# Autodesk Inventor assembly: Elevator
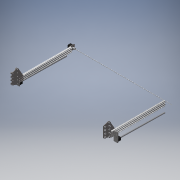
[picture p0: Inventor's stored thumbnail of the model, 180x180]
Saved by Autodesk Inventor 2017 (Build 210142000, 142)
## iProperties
Created: 2016-12-12
Part Number: Elevator
Document SubType Name: Assembly
Designer: umr
Author: umr
## Documents named in this file (21)
- D:\SeniorProject\Models2\Gantry\GantryDown.iam
- D:\SeniorProject\Models2\Gantry\Gantry Plate.ipt
- D:\SeniorProject\Models2\Gantry\M5 Screw with Tee Nut.iam
- D:\SeniorProject\Models2\Gantry\Solid Wheel with Eccentric Spacer Assembly.iam
- D:\SeniorProject\Models2\Gantry\L_Fixer.ipt
- D:\SeniorProject\Models2\Gantry\ScrewDriver.ipt
- D:\SeniorProject\Models2\Gantry\MotorFixer.ipt
- D:\SeniorProject\Models2\Gantry\Elevator Track.ipt
- D:\SeniorProject\Models2\Gantry\Motor.ipt
- D:\SeniorProject\Models2\Gantry\Motor Mount Plate.ipt
- D:\SeniorProject\Models2\Gantry\Driveshaft.ipt
- D:\SeniorProject\Models2\Gantry\5mm x 5mm Flexible Coupling.ipt
- D:\SeniorProject\Models2\Gantry\GT2 20 Tooth Pulley.ipt
- D:\SeniorProject\Models2\Gantry\Gantry Plate_MIR.ipt
- D:\SeniorProject\Models2\Gantry\M5 Screw with Tee Nut_MIR.iam
- D:\SeniorProject\Models2\Gantry\Solid Wheel with Eccentric Spacer Assembly_MIR.iam
- D:\SeniorProject\Models2\Gantry\L_Fixer_MIR.ipt
- D:\SeniorProject\Models2\Gantry\ScrewDriver_MIR.ipt
- D:\SeniorProject\Models2\Gantry\MotorFixer_MIR.ipt
- D:\SeniorProject\Models2\Gantry\Elevator Track_MIR.ipt
- D:\SeniorProject\Models2\Gantry\Motor_MIR.ipt
## Components (62 placed, 20 different names)
1. Gantry Plate:1 — Mate:1, Mate:2, Mate:3, Mate:4, Mate:5, Mate:6, Mate:7, Mate:8, Mate:9, Mate:11, Mate:12, Mate:13, Mate:14, Mate:16, Mate:17, Mate:18, Mate:21, Mate:22, Mate:26, Mate:27, Mate:28, Mate:29, Mate:30, Mate:31, Mate:32, Mate:33, Mate:34, Mate:35, Mate:36, Mate:37, Mate:38, Mate:39, Mate:40, Mate:41, Mate:42, Mate:43
2. M5 Screw with Tee Nut:1 [sub-assembly] — Mate:1, Mate:2
3. M5 Screw with Tee Nut:2 [sub-assembly] — Mate:3, Mate:14
4. M5 Screw with Tee Nut:3 [sub-assembly] — Mate:4, Mate:11
5. M5 Screw with Tee Nut:4 [sub-assembly] — Mate:5, Mate:18
6. M5 Screw with Tee Nut:5 [sub-assembly] — Mate:6, Mate:12
7. M5 Screw with Tee Nut:6 [sub-assembly] — Mate:7, Mate:13, Mate:56, Mate:57
8. M5 Screw with Tee Nut:7 [sub-assembly] — Mate:8, Mate:16
9. M5 Screw with Tee Nut:8 [sub-assembly] — Mate:9, Mate:17, Mate:58
10. M5 Screw with Tee Nut:9 [sub-assembly] — Mate:21, Mate:22
11. Solid Wheel with Eccentric Spacer Assembly:1 [sub-assembly] — Mate:29, Mate:43
12. Solid Wheel with Eccentric Spacer Assembly:2 [sub-assembly] — Mate:26, Mate:40
13. Solid Wheel with Eccentric Spacer Assembly:3 [sub-assembly] — Mate:27, Mate:39
14. Solid Wheel with Eccentric Spacer Assembly:4 [sub-assembly] — Mate:28, Mate:41
15. Solid Wheel with Eccentric Spacer Assembly:5 [sub-assembly] — Mate:30, Mate:42
16. Solid Wheel with Eccentric Spacer Assembly:6 [sub-assembly] — Mate:31, Mate:35
17. Solid Wheel with Eccentric Spacer Assembly:7 [sub-assembly] — Mate:32, Mate:36
18. Solid Wheel with Eccentric Spacer Assembly:8 [sub-assembly] — Mate:33, Mate:37
19. Solid Wheel with Eccentric Spacer Assembly:10 [sub-assembly] — Mate:34, Mate:38
20. L_Fixer:1 — Mate:44, Mate:45, Mate:46, Mate:47, Mate:48, Mate:49, Mate:69, Mate:70, Mate:71
21. M5 Screw with Tee Nut:10 [sub-assembly] — Mate:44, Mate:47, Mate:67
22. M5 Screw with Tee Nut:11 [sub-assembly] — Mate:45, Mate:48, Mate:68
23. M5 Screw with Tee Nut:12 [sub-assembly] — Mate:46, Mate:49, Mate:66
24. ScrewDriver:1 — Mate:72, Mate:73
25. MotorFixer:1 — Mate:69, Mate:70, Mate:71, Mate:74
26. Elevator Track:1 — Mate:56, Mate:57, Mate:58, Mate:66, Mate:67, Mate:68, Mate:82, Mate:83, Mate:85, Mate:86, Mate:87, Flush:2
27. Motor:1 — Mate:72, Mate:73, Mate:74
28. Motor Mount Plate:1 — Mate:88, Mate:89, Mate:90, Mate:91, Mate:92, Mate:93, Mate:94, Mate:95
29. M5 Screw with Tee Nut:15 [sub-assembly] — Mate:82, Mate:83, Mate:89, Mate:91
30. M5 Screw with Tee Nut:16 [sub-assembly] — Mate:85, Mate:90, Flush:2
31. M5 Screw with Tee Nut:17 [sub-assembly] — Mate:86, Mate:87, Mate:88
32. Motor:2 — Mate:92, Mate:93, Mate:94, Mate:95, Mate:96, Mate:98, Mate:99, Mate:100
33. 5mm x 5mm Flexible Coupling:1 — Mate:96, Mate:97, Mate:101
34. Driveshaft:1 — Mate:97, Mate:98
35. GT2 20 Tooth Pulley:1 — Mate:99, Mate:100, Mate:101
36. Gantry Plate_MIR:1 — Mate:102, Mate:103, Mate:104, Mate:105, Mate:106, Mate:107, Mate:108, Mate:109, Mate:110, Mate:111, Mate:112, Mate:113, Mate:114, Mate:115, Mate:116, Mate:117, Mate:118, Mate:119, Mate:120, Mate:121, Mate:122, Mate:123, Mate:124, Mate:125, Mate:126, Mate:127, Mate:128, Mate:129, Mate:130, Mate:131, Mate:132, Mate:133, Mate:134, Mate:135, Mate:136, Mate:137
37. M5 Screw with Tee Nut_MIR:1 [sub-assembly] — Mate:102, Mate:103
38. M5 Screw with Tee Nut_MIR:2 [sub-assembly] — Mate:104, Mate:105
39. M5 Screw with Tee Nut_MIR:3 [sub-assembly] — Mate:106, Mate:107
40. M5 Screw with Tee Nut_MIR:4 [sub-assembly] — Mate:108, Mate:109
41. M5 Screw with Tee Nut_MIR:5 [sub-assembly] — Mate:110, Mate:111
42. M5 Screw with Tee Nut_MIR:6 [sub-assembly] — Mate:112, Mate:113, Mate:157, Mate:158
43. M5 Screw with Tee Nut_MIR:7 [sub-assembly] — Mate:114, Mate:115
44. M5 Screw with Tee Nut_MIR:8 [sub-assembly] — Mate:116, Mate:117, Mate:156
45. M5 Screw with Tee Nut_MIR:9 [sub-assembly] — Mate:118, Mate:119
46. Solid Wheel with Eccentric Spacer Assembly_MIR:1 [sub-assembly] — Mate:120, Mate:121
47. Solid Wheel with Eccentric Spacer Assembly_MIR:2 [sub-assembly] — Mate:122, Mate:123
48. Solid Wheel with Eccentric Spacer Assembly_MIR:3 [sub-assembly] — Mate:124, Mate:125
49. Solid Wheel with Eccentric Spacer Assembly_MIR:4 [sub-assembly] — Mate:126, Mate:127
50. Solid Wheel with Eccentric Spacer Assembly_MIR:5 [sub-assembly] — Mate:128, Mate:129
51. Solid Wheel with Eccentric Spacer Assembly_MIR:6 [sub-assembly] — Mate:130, Mate:131
52. Solid Wheel with Eccentric Spacer Assembly_MIR:7 [sub-assembly] — Mate:132, Mate:133
53. Solid Wheel with Eccentric Spacer Assembly_MIR:8 [sub-assembly] — Mate:134, Mate:135
54. Solid Wheel with Eccentric Spacer Assembly_MIR:9 [sub-assembly] — Mate:136, Mate:137
55. L_Fixer_MIR:1 — Mate:138, Mate:139, Mate:140, Mate:141, Mate:142, Mate:143, Mate:150, Mate:151, Mate:152
56. M5 Screw with Tee Nut_MIR:10 [sub-assembly] — Mate:138, Mate:139, Mate:154
57. M5 Screw with Tee Nut_MIR:11 [sub-assembly] — Mate:140, Mate:141, Mate:153
58. M5 Screw with Tee Nut_MIR:12 [sub-assembly] — Mate:142, Mate:143, Mate:155
59. ScrewDriver_MIR:1 — Mate:167, Mate:168
60. MotorFixer_MIR:1 — Mate:150, Mate:151, Mate:152, Mate:166
61. Elevator Track_MIR:1 — Mate:153, Mate:154, Mate:155, Mate:156, Mate:157, Mate:158
62. Motor_MIR:1 — Mate:166, Mate:167, Mate:168
## Relationships (128: Mate 127, Flush 1)
- Mate:1: Gantry Plate:1 ↔ M5 Screw with Tee Nut:1
- Mate:2: Gantry Plate:1 ↔ M5 Screw with Tee Nut:1
- Mate:3: Gantry Plate:1 ↔ M5 Screw with Tee Nut:2
- Mate:4: Gantry Plate:1 ↔ M5 Screw with Tee Nut:3
- Mate:5: Gantry Plate:1 ↔ M5 Screw with Tee Nut:4
- Mate:6: Gantry Plate:1 ↔ M5 Screw with Tee Nut:5
- Mate:7: Gantry Plate:1 ↔ M5 Screw with Tee Nut:6
- Mate:8: Gantry Plate:1 ↔ M5 Screw with Tee Nut:7
- Mate:9: Gantry Plate:1 ↔ M5 Screw with Tee Nut:8
- Mate:11: Gantry Plate:1 ↔ M5 Screw with Tee Nut:3
- Mate:12: Gantry Plate:1 ↔ M5 Screw with Tee Nut:5
- Mate:13: Gantry Plate:1 ↔ M5 Screw with Tee Nut:6
- Mate:14: Gantry Plate:1 ↔ M5 Screw with Tee Nut:2
- Mate:16: Gantry Plate:1 ↔ M5 Screw with Tee Nut:7
- Mate:17: Gantry Plate:1 ↔ M5 Screw with Tee Nut:8
- Mate:18: Gantry Plate:1 ↔ M5 Screw with Tee Nut:4
- Mate:21: Gantry Plate:1 ↔ M5 Screw with Tee Nut:9
- Mate:22: Gantry Plate:1 ↔ M5 Screw with Tee Nut:9
- Mate:26: Gantry Plate:1 ↔ Solid Wheel with Eccentric Spacer Assembly:2
- Mate:27: Gantry Plate:1 ↔ Solid Wheel with Eccentric Spacer Assembly:3
- Mate:28: Gantry Plate:1 ↔ Solid Wheel with Eccentric Spacer Assembly:4
- Mate:29: Gantry Plate:1 ↔ Solid Wheel with Eccentric Spacer Assembly:1
- Mate:30: Gantry Plate:1 ↔ Solid Wheel with Eccentric Spacer Assembly:5
- Mate:31: Gantry Plate:1 ↔ Solid Wheel with Eccentric Spacer Assembly:6
- Mate:32: Gantry Plate:1 ↔ Solid Wheel with Eccentric Spacer Assembly:7
- Mate:33: Gantry Plate:1 ↔ Solid Wheel with Eccentric Spacer Assembly:8
- Mate:34: Gantry Plate:1 ↔ Solid Wheel with Eccentric Spacer Assembly:10
- Mate:35: Gantry Plate:1 ↔ Solid Wheel with Eccentric Spacer Assembly:6
- Mate:36: Gantry Plate:1 ↔ Solid Wheel with Eccentric Spacer Assembly:7
- Mate:37: Gantry Plate:1 ↔ Solid Wheel with Eccentric Spacer Assembly:8
- Mate:38: Gantry Plate:1 ↔ Solid Wheel with Eccentric Spacer Assembly:10
- Mate:39: Gantry Plate:1 ↔ Solid Wheel with Eccentric Spacer Assembly:3
- Mate:40: Gantry Plate:1 ↔ Solid Wheel with Eccentric Spacer Assembly:2
- Mate:41: Gantry Plate:1 ↔ Solid Wheel with Eccentric Spacer Assembly:4
- Mate:42: Gantry Plate:1 ↔ Solid Wheel with Eccentric Spacer Assembly:5
- Mate:43: Gantry Plate:1 ↔ Solid Wheel with Eccentric Spacer Assembly:1
- Mate:44: L_Fixer:1 ↔ M5 Screw with Tee Nut:10
- Mate:45: L_Fixer:1 ↔ M5 Screw with Tee Nut:11
- Mate:46: L_Fixer:1 ↔ M5 Screw with Tee Nut:12
- Mate:47: L_Fixer:1 ↔ M5 Screw with Tee Nut:10
- Mate:48: L_Fixer:1 ↔ M5 Screw with Tee Nut:11
- Mate:49: L_Fixer:1 ↔ M5 Screw with Tee Nut:12
- Mate:56: M5 Screw with Tee Nut:6 ↔ Elevator Track:1
- Mate:57: M5 Screw with Tee Nut:6 ↔ Elevator Track:1
- Mate:58: M5 Screw with Tee Nut:8 ↔ Elevator Track:1
- Mate:66: M5 Screw with Tee Nut:12 ↔ Elevator Track:1
- Mate:67: M5 Screw with Tee Nut:10 ↔ Elevator Track:1
- Mate:68: M5 Screw with Tee Nut:11 ↔ Elevator Track:1
- Mate:69: L_Fixer:1 ↔ MotorFixer:1
- Mate:70: L_Fixer:1 ↔ MotorFixer:1
- Mate:71: L_Fixer:1 ↔ MotorFixer:1
- Mate:72: ScrewDriver:1 ↔ Motor:1
- Mate:73: ScrewDriver:1 ↔ Motor:1
- Mate:74: MotorFixer:1 ↔ Motor:1
- Mate:82 (0.5 mm): Elevator Track:1 ↔ M5 Screw with Tee Nut:15
- Mate:83 (1 mm): Elevator Track:1 ↔ M5 Screw with Tee Nut:15
- Mate:85 (1 mm): Elevator Track:1 ↔ M5 Screw with Tee Nut:16
- Mate:86 (0.5 mm): Elevator Track:1 ↔ M5 Screw with Tee Nut:17
- Mate:87 (1 mm): Elevator Track:1 ↔ M5 Screw with Tee Nut:17
- Mate:88: Motor Mount Plate:1 ↔ M5 Screw with Tee Nut:17
- Mate:89: Motor Mount Plate:1 ↔ M5 Screw with Tee Nut:15
- Mate:90: Motor Mount Plate:1 ↔ M5 Screw with Tee Nut:16
- Mate:91: Motor Mount Plate:1 ↔ M5 Screw with Tee Nut:15
- Flush:2 (5 mm): Elevator Track:1 ↔ M5 Screw with Tee Nut:16
- Mate:92: Motor Mount Plate:1 ↔ Motor:2
- Mate:93: Motor Mount Plate:1 ↔ Motor:2
- Mate:94: Motor Mount Plate:1 ↔ Motor:2
- Mate:95: Motor Mount Plate:1 ↔ Motor:2
- Mate:96: Motor:2 ↔ 5mm x 5mm Flexible Coupling:1
- Mate:97: 5mm x 5mm Flexible Coupling:1 ↔ Driveshaft:1
- Mate:98: Motor:2 ↔ Driveshaft:1
- Mate:99: Motor:2 ↔ GT2 20 Tooth Pulley:1
- Mate:100: Motor:2 ↔ GT2 20 Tooth Pulley:1
- Mate:101: 5mm x 5mm Flexible Coupling:1 ↔ GT2 20 Tooth Pulley:1
- Mate:102: Gantry Plate_MIR:1 ↔ M5 Screw with Tee Nut_MIR:1
- Mate:103: Gantry Plate_MIR:1 ↔ M5 Screw with Tee Nut_MIR:1
- Mate:104: Gantry Plate_MIR:1 ↔ M5 Screw with Tee Nut_MIR:2
- Mate:105: Gantry Plate_MIR:1 ↔ M5 Screw with Tee Nut_MIR:2
- Mate:106: Gantry Plate_MIR:1 ↔ M5 Screw with Tee Nut_MIR:3
- Mate:107: Gantry Plate_MIR:1 ↔ M5 Screw with Tee Nut_MIR:3
- Mate:108: Gantry Plate_MIR:1 ↔ M5 Screw with Tee Nut_MIR:4
- Mate:109: Gantry Plate_MIR:1 ↔ M5 Screw with Tee Nut_MIR:4
- Mate:110: Gantry Plate_MIR:1 ↔ M5 Screw with Tee Nut_MIR:5
- Mate:111: Gantry Plate_MIR:1 ↔ M5 Screw with Tee Nut_MIR:5
- Mate:112: Gantry Plate_MIR:1 ↔ M5 Screw with Tee Nut_MIR:6
- Mate:113: Gantry Plate_MIR:1 ↔ M5 Screw with Tee Nut_MIR:6
- Mate:114: Gantry Plate_MIR:1 ↔ M5 Screw with Tee Nut_MIR:7
- Mate:115: Gantry Plate_MIR:1 ↔ M5 Screw with Tee Nut_MIR:7
- Mate:116: Gantry Plate_MIR:1 ↔ M5 Screw with Tee Nut_MIR:8
- Mate:117: Gantry Plate_MIR:1 ↔ M5 Screw with Tee Nut_MIR:8
- Mate:118: Gantry Plate_MIR:1 ↔ M5 Screw with Tee Nut_MIR:9
- Mate:119: Gantry Plate_MIR:1 ↔ M5 Screw with Tee Nut_MIR:9
- Mate:120: Gantry Plate_MIR:1 ↔ Solid Wheel with Eccentric Spacer Assembly_MIR:1
- Mate:121: Gantry Plate_MIR:1 ↔ Solid Wheel with Eccentric Spacer Assembly_MIR:1
- Mate:122: Gantry Plate_MIR:1 ↔ Solid Wheel with Eccentric Spacer Assembly_MIR:2
- Mate:123: Gantry Plate_MIR:1 ↔ Solid Wheel with Eccentric Spacer Assembly_MIR:2
- Mate:124: Gantry Plate_MIR:1 ↔ Solid Wheel with Eccentric Spacer Assembly_MIR:3
- Mate:125: Gantry Plate_MIR:1 ↔ Solid Wheel with Eccentric Spacer Assembly_MIR:3
- Mate:126: Gantry Plate_MIR:1 ↔ Solid Wheel with Eccentric Spacer Assembly_MIR:4
- Mate:127: Gantry Plate_MIR:1 ↔ Solid Wheel with Eccentric Spacer Assembly_MIR:4
- Mate:128: Gantry Plate_MIR:1 ↔ Solid Wheel with Eccentric Spacer Assembly_MIR:5
- Mate:129: Gantry Plate_MIR:1 ↔ Solid Wheel with Eccentric Spacer Assembly_MIR:5
- Mate:130: Gantry Plate_MIR:1 ↔ Solid Wheel with Eccentric Spacer Assembly_MIR:6
- Mate:131: Gantry Plate_MIR:1 ↔ Solid Wheel with Eccentric Spacer Assembly_MIR:6
- Mate:132: Gantry Plate_MIR:1 ↔ Solid Wheel with Eccentric Spacer Assembly_MIR:7
- Mate:133: Gantry Plate_MIR:1 ↔ Solid Wheel with Eccentric Spacer Assembly_MIR:7
- Mate:134: Gantry Plate_MIR:1 ↔ Solid Wheel with Eccentric Spacer Assembly_MIR:8
- Mate:135: Gantry Plate_MIR:1 ↔ Solid Wheel with Eccentric Spacer Assembly_MIR:8
- Mate:136: Gantry Plate_MIR:1 ↔ Solid Wheel with Eccentric Spacer Assembly_MIR:9
- Mate:137: Gantry Plate_MIR:1 ↔ Solid Wheel with Eccentric Spacer Assembly_MIR:9
- Mate:138: L_Fixer_MIR:1 ↔ M5 Screw with Tee Nut_MIR:10
- Mate:139: L_Fixer_MIR:1 ↔ M5 Screw with Tee Nut_MIR:10
- Mate:140: L_Fixer_MIR:1 ↔ M5 Screw with Tee Nut_MIR:11
- Mate:141: L_Fixer_MIR:1 ↔ M5 Screw with Tee Nut_MIR:11
- Mate:142: L_Fixer_MIR:1 ↔ M5 Screw with Tee Nut_MIR:12
- Mate:143: L_Fixer_MIR:1 ↔ M5 Screw with Tee Nut_MIR:12
- Mate:150: L_Fixer_MIR:1 ↔ MotorFixer_MIR:1
- Mate:151: L_Fixer_MIR:1 ↔ MotorFixer_MIR:1
- Mate:152: L_Fixer_MIR:1 ↔ MotorFixer_MIR:1
- Mate:153: M5 Screw with Tee Nut_MIR:11 ↔ Elevator Track_MIR:1
- Mate:154: M5 Screw with Tee Nut_MIR:10 ↔ Elevator Track_MIR:1
- Mate:155: M5 Screw with Tee Nut_MIR:12 ↔ Elevator Track_MIR:1
- Mate:156: M5 Screw with Tee Nut_MIR:8 ↔ Elevator Track_MIR:1
- Mate:157: M5 Screw with Tee Nut_MIR:6 ↔ Elevator Track_MIR:1
- Mate:158: M5 Screw with Tee Nut_MIR:6 ↔ Elevator Track_MIR:1
- Mate:166: MotorFixer_MIR:1 ↔ Motor_MIR:1
- Mate:167: ScrewDriver_MIR:1 ↔ Motor_MIR:1
- Mate:168: ScrewDriver_MIR:1 ↔ Motor_MIR:1
